# Autodesk Inventor assembly: Body Assembly
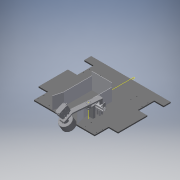
[picture p0: Inventor's stored thumbnail of the model, 180x180]
Saved by Autodesk Inventor 2019 (Build 230136000, 136)
## iProperties
Created: 2019-10-15
Part Number: Body Assembly
Document SubType Name: Assembly
Designer: User
Author: User
## Documents named in this file (14)
- C:\Robotics\CAD\2019-20_CAD\Collection\Body Assembly.iam
- C:\Robotics\CAD\2019-20_CAD\Collection\U-Part Gen 2.ipt
- C:\Robotics\CAD\COTSParts\Actobotics\545 parts\545364 assembly.ipt
- C:\Robotics\CAD\2019-20_CAD\Collection\wheel arm stand off.ipt
- C:\Robotics\CAD\2019-20_CAD\Drive Train\Gen 2.0 rev mecanums base plate.ipt
- C:\Robotics\CAD\2019-20_CAD\Collection\arm assembaly.iam
- C:\Robotics\CAD\COTSParts\Vex\2-Wire_Motor_393_276-2177.iam
- C:\Robotics\CAD\COTSParts\Wheels\2.5inFoamWheel250TMD.ipt
- C:\Robotics\CAD\2019-20_CAD\Collection\vex motor adaptor to tetrix.ipt
- C:\Robotics\CAD\COTSParts\Bearings - AndyMark\Bearing 250 ID 500 OD flanged.ipt
- C:\Robotics\CAD\COTSParts\Bosch Extrusion\Bosch 20x20 - 1.5 Part.Shoot.ipt
- C:\Robotics\CAD\COTSParts\Bosch Extrusion\Bosch 20x20 - 4.5 Part.Shoot.ipt
- C:\Robotics\CAD\2019-20_CAD\Collection\spring tab for on 20x20.ipt
- C:\Robotics\CAD\2019-20_CAD\Collection\stop for on 20x20.ipt
## Components (13 placed, 12 different names)
1. U-Part Gen 2:1 — Mate:19, Flush:8, Mate:23, Flush:9, Flush:10, Mate:36, Mate:40
2. 545364 assembly:2 — Mate:17, Mate:18, Mate:20
3. wheel arm stand off:2 — Mate:17, Mate:18, Mate:21, Mate:22, Mate:23, Flush:10, Mate:38
4. Gen 2.0 rev mecanums base plate:1 — Mate:19, Flush:8, Mate:21, Flush:9, Flush:11, Mate:34
5. arm assembaly:1 [sub-assembly] — Mate:20, Mate:22, Mate:24, Mate:25, Mate:26, Mate:28, Mate:32
6. 2-Wire_Motor_393_276-2177:1 [sub-assembly] — Mate:24, Mate:25, Mate:26, Mate:27
7. vex motor adaptor to tetrix:1 — Mate:27, Mate:28, Mate:29, Insert:1, Mate:30, Mate:31
8. 2.5inFoamWheel250TMD:1 — Mate:29, Insert:1, Mate:30
9. Bearing 250 ID 500 OD flanged:1 — Mate:31, Mate:32
10. Bosch 20x20 - 1.5 Part.Shoot:2 — Mate:34, Mate:35, Flush:12, Flush:13, Mate:38
11. Bosch 20x20 - 4.5 Part.Shoot:1 — Mate:35, Flush:12, Mate:36, Flush:13, Mate:39, Flush:14, Flush:16
12. spring tab for on arm:1 — Mate:39, Mate:40, Flush:14, Flush:15, Flush:17
13. spring tab for on arm:2 — Flush:15, Flush:16, Flush:17
## Relationships (33: Mate 22, Flush 10, Insert 1)
- Mate:17: 545364 assembly:2 ↔ wheel arm stand off:2
- Mate:18: 545364 assembly:2 ↔ wheel arm stand off:2
- Mate:19: U-Part Gen 2:1 ↔ Gen 2.0 rev mecanums base plate:1
- Flush:8 (203.2 mm): U-Part Gen 2:1 ↔ Gen 2.0 rev mecanums base plate:1
- Mate:20: 545364 assembly:2 ↔ arm assembaly:1
- Mate:21: wheel arm stand off:2 ↔ Gen 2.0 rev mecanums base plate:1
- Mate:22: wheel arm stand off:2 ↔ arm assembaly:1
- Mate:23 (4.7625 mm): U-Part Gen 2:1 ↔ wheel arm stand off:2
- Flush:9 (-110.1725 mm): U-Part Gen 2:1 ↔ Gen 2.0 rev mecanums base plate:1
- Flush:10 (-121.1072 mm): U-Part Gen 2:1 ↔ wheel arm stand off:2
- Mate:24: arm assembaly:1 ↔ 2-Wire_Motor_393_276-2177:1
- Mate:25: arm assembaly:1 ↔ 2-Wire_Motor_393_276-2177:1
- Mate:26: arm assembaly:1 ↔ 2-Wire_Motor_393_276-2177:1
- Mate:27: 2-Wire_Motor_393_276-2177:1 ↔ vex motor adaptor to tetrix:1
- Mate:28: arm assembaly:1 ↔ vex motor adaptor to tetrix:1
- Mate:29: vex motor adaptor to tetrix:1 ↔ 2.5inFoamWheel250TMD:1
- Insert:1: vex motor adaptor to tetrix:1 ↔ 2.5inFoamWheel250TMD:1
- Mate:30: vex motor adaptor to tetrix:1 ↔ 2.5inFoamWheel250TMD:1
- Flush:11 (-215.9 mm): Gen 2.0 rev mecanums base plate:1
- Mate:31: vex motor adaptor to tetrix:1 ↔ Bearing 250 ID 500 OD flanged:1
- Mate:32: arm assembaly:1 ↔ Bearing 250 ID 500 OD flanged:1
- Mate:34: Gen 2.0 rev mecanums base plate:1 ↔ Bosch 20x20 - 1.5 Part.Shoot:2
- Mate:35: Bosch 20x20 - 1.5 Part.Shoot:2 ↔ Bosch 20x20 - 4.5 Part.Shoot:1
- Flush:12: Bosch 20x20 - 1.5 Part.Shoot:2 ↔ Bosch 20x20 - 4.5 Part.Shoot:1
- Mate:36: U-Part Gen 2:1 ↔ Bosch 20x20 - 4.5 Part.Shoot:1
- Flush:13 (15.4051 mm): Bosch 20x20 - 1.5 Part.Shoot:2 ↔ Bosch 20x20 - 4.5 Part.Shoot:1
- Mate:38 (18.1102 mm): wheel arm stand off:2 ↔ Bosch 20x20 - 1.5 Part.Shoot:2
- Mate:39: Bosch 20x20 - 4.5 Part.Shoot:1 ↔ spring tab for on arm:1
- Mate:40: U-Part Gen 2:1 ↔ spring tab for on arm:1
- Flush:14 (3.65 mm): Bosch 20x20 - 4.5 Part.Shoot:1 ↔ spring tab for on arm:1
- Flush:15: spring tab for on arm:1 ↔ spring tab for on arm:2
- Flush:16: Bosch 20x20 - 4.5 Part.Shoot:1 ↔ spring tab for on arm:2
- Flush:17: spring tab for on arm:1 ↔ spring tab for on arm:2
